# Autodesk Inventor assembly: RightNEXUSAdapterDriveTrain2.0
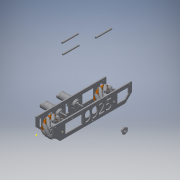
[picture p0: Inventor's stored thumbnail of the model, 180x180]
Saved by Autodesk Inventor 2017 (Build 210142000, 142)
## iProperties
Created: 2017-08-12
Part Number: RightNEXUSAdapterDriveTrain2.0
Document SubType Name: Assembly
Designer: User
Author: User
## Documents named in this file (13)
- C:\Robotics\CAD\2016-17_CAD\DriveTrain\RightNEXUSAdapterDriveTrain2.0.iam
- C:\Robotics\CAD\2016-17_CAD\DriveTrain\DriveTrainPlate2.0RightInside.ipt
- C:\Robotics\CAD\2016-17_CAD\DriveTrain\DriveTrainPlate2.0RightOutside.iam
- C:\Robotics\CAD\2016-17_CAD\DriveTrain\drive train standoff.ipt
- C:\Robotics\CAD\COTSParts\Motors\Andymark 2964  NeveRest 40 Motor.ipt
- C:\Robotics\CAD\COTSParts\Wheels\AndyMark Mecanum Wheels\100mm Aluminum Mecanum wheels.ipt
- C:\Robotics\CAD\COTSParts\Actobotics\545 parts\545556.ipt
- C:\Robotics\CAD\COTSParts\Actobotics\545 parts\545456.ipt
- C:\Robotics\CAD\COTSParts\Actobotics\535 parts\535198.ipt
- C:\Robotics\CAD\COTSParts\Actobotics\615 parts\615102.ipt
- C:\Robotics\CAD\COTSParts\Actobotics\634 parts\634080.ipt
- C:\Robotics\CAD\COTSParts\Tetrix\tetrix-motor-mounts-1.snapshot.1\Tetrex 2pc motor mount.ipt
- C:\Robotics\CAD\COTSParts\Actobotics\collar.ipt
## Components (35 placed, 12 different names)
1. DriveTrainPlate2.0RightInside:1 — Mate:23, Mate:24, Flush:1, Mate:34, Mate:35, Mate:72, Mate:73, Mate:74, Mate:75, Mate:76, Mate:77
2. DriveTrainPlate2.0RightOutside:1 [sub-assembly] — Mate:63, Mate:64, Mate:65
3. drive train standoff:1
4. drive train standoff:2
5. drive train standoff:3
6. Andymark 2964  NeveRest 40 Motor:1 — Insert:6, Mate:67, Mate:69, Mate:77
7. Andymark 2964  NeveRest 40 Motor:2 — Insert:5, Mate:66, Mate:71, Mate:74
8. 100mm Aluminum Mecanum wheels:1 — Mate:7, Mate:22, Mate:44
9. 100mm Aluminum Mecanum wheels:2 — Mate:16, Mate:25, Mate:37
10. 545556:1 — Mate:56, Mate:57, Mate:58
11. 545556:2 — Mate:29, Mate:30, Mate:33
12. 545556:3 — Insert:3, Mate:10, Mate:19
13. 545556:4 — Mate:60, Mate:61, Mate:62
14. 545456:1 — Mate:36, Mate:37, Mate:61
15. 545456:2 — Mate:25, Mate:26, Mate:28
16. 545456:3 — Mate:44, Mate:45, Mate:57
17. 545456:4 — Mate:7, Mate:8, Mate:9, Mate:21
18. 535198:1 — Mate:43, Mate:59
19. 535198:2 — Mate:51, Mate:53, Mate:63
20. 535198:3 — Insert:2, Mate:12, Mate:31, Insert:4, Mate:35
21. 535198:4 — Mate:11, Mate:17, Mate:24
22. 615102:1 — Mate:66, Mate:70
23. 615102:2 — Mate:27, Mate:28, Mate:30
24. 615102:3 — Mate:8, Mate:9, Insert:3, Mate:20
25. 615102:4 — Mate:67, Mate:68
26. 545556:5 — Mate:70, Mate:71
27. 545556:6 — Mate:68, Mate:69
28. 634080:1 — Mate:17, Mate:18, Mate:19, Mate:20, Mate:21, Mate:22, Flush:1, Mate:45, Mate:51, Mate:55, Mate:56, Mate:64
29. 634080:2 — Mate:12, Mate:16, Mate:26, Mate:27, Mate:29, Mate:31, Mate:32, Insert:4, Mate:36, Mate:41, Mate:43, Mate:60, Mate:65
30. Tetrex 2pc motor mount:1 — Insert:5, Mate:72, Mate:73
31. Tetrex 2pc motor mount:2 — Insert:6, Mate:75, Mate:76
32. collar:1 — Insert:2, Mate:32, Mate:33, Mate:34
33. collar:2 — Mate:41, Mate:59, Mate:62
34. collar:3 — Mate:53, Mate:55, Mate:58
35. collar:4 — Mate:10, Mate:11, Mate:18, Mate:23
## Relationships (63: Mate 57, Insert 5, Flush 1)
- Insert:2: 535198:3 ↔ collar:1
- Mate:7: 100mm Aluminum Mecanum wheels:1 ↔ 545456:4
- Mate:8: 545456:4 ↔ 615102:3
- Mate:9: 545456:4 ↔ 615102:3
- Insert:3: 545556:3 ↔ 615102:3
- Mate:10: 545556:3 ↔ collar:4
- Mate:11: 535198:4 ↔ collar:4
- Mate:12: 535198:3 ↔ 634080:2
- Mate:16: 100mm Aluminum Mecanum wheels:2 ↔ 634080:2
- Mate:17: 535198:4 ↔ 634080:1
- Mate:18: 634080:1 ↔ collar:4
- Mate:19: 545556:3 ↔ 634080:1
- Mate:20: 615102:3 ↔ 634080:1
- Mate:21: 545456:4 ↔ 634080:1
- Mate:22: 100mm Aluminum Mecanum wheels:1 ↔ 634080:1
- Mate:23: DriveTrainPlate2.0RightInside:1 ↔ collar:4
- Mate:24: DriveTrainPlate2.0RightInside:1 ↔ 535198:4
- Flush:1: DriveTrainPlate2.0RightInside:1 ↔ 634080:1
- Mate:25: 100mm Aluminum Mecanum wheels:2 ↔ 545456:2
- Mate:26: 545456:2 ↔ 634080:2
- Mate:27: 615102:2 ↔ 634080:2
- Mate:28: 545456:2 ↔ 615102:2
- Mate:29: 545556:2 ↔ 634080:2
- Mate:30: 545556:2 ↔ 615102:2
- Mate:31: 535198:3 ↔ 634080:2
- Mate:32: 634080:2 ↔ collar:1
- Mate:33: 545556:2 ↔ collar:1
- Insert:4: 535198:3 ↔ 634080:2
- Mate:34: DriveTrainPlate2.0RightInside:1 ↔ collar:1
- Mate:35: DriveTrainPlate2.0RightInside:1 ↔ 535198:3
- Mate:36: 545456:1 ↔ 634080:2
- Mate:37: 100mm Aluminum Mecanum wheels:2 ↔ 545456:1
- Mate:41: 634080:2 ↔ collar:2
- Mate:43: 535198:1 ↔ 634080:2
- Mate:44: 100mm Aluminum Mecanum wheels:1 ↔ 545456:3
- Mate:45: 545456:3 ↔ 634080:1
- Mate:51: 535198:2 ↔ 634080:1
- Mate:53: 535198:2 ↔ collar:3
- Mate:55: 634080:1 ↔ collar:3
- Mate:56: 545556:1 ↔ 634080:1
- Mate:57: 545556:1 ↔ 545456:3
- Mate:58: 545556:1 ↔ collar:3
- Mate:59: 535198:1 ↔ collar:2
- Mate:60: 545556:4 ↔ 634080:2
- Mate:61: 545556:4 ↔ 545456:1
- Mate:62: 545556:4 ↔ collar:2
- Mate:63: DriveTrainPlate2.0RightOutside:1 ↔ 535198:2
- Mate:64: DriveTrainPlate2.0RightOutside:1 ↔ 634080:1
- Mate:65: DriveTrainPlate2.0RightOutside:1 ↔ 634080:2
- Insert:5: Andymark 2964  NeveRest 40 Motor:2 ↔ Tetrex 2pc motor mount:1
- Mate:66: Andymark 2964  NeveRest 40 Motor:2 ↔ 615102:1
- Insert:6: Andymark 2964  NeveRest 40 Motor:1 ↔ Tetrex 2pc motor mount:2
- Mate:67: Andymark 2964  NeveRest 40 Motor:1 ↔ 615102:4
- Mate:68: 615102:4 ↔ 545556:6
- Mate:69: Andymark 2964  NeveRest 40 Motor:1 ↔ 545556:6
- Mate:70: 615102:1 ↔ 545556:5
- Mate:71: Andymark 2964  NeveRest 40 Motor:2 ↔ 545556:5
- Mate:72: DriveTrainPlate2.0RightInside:1 ↔ Tetrex 2pc motor mount:1
- Mate:73: DriveTrainPlate2.0RightInside:1 ↔ Tetrex 2pc motor mount:1
- Mate:74: DriveTrainPlate2.0RightInside:1 ↔ Andymark 2964  NeveRest 40 Motor:2
- Mate:75: DriveTrainPlate2.0RightInside:1 ↔ Tetrex 2pc motor mount:2
- Mate:76: DriveTrainPlate2.0RightInside:1 ↔ Tetrex 2pc motor mount:2
- Mate:77: DriveTrainPlate2.0RightInside:1 ↔ Andymark 2964  NeveRest 40 Motor:1
